# Autodesk Inventor assembly: CockpitLED
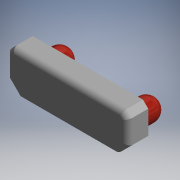
[picture p0: Inventor's stored thumbnail of the model, 180x180]
Saved by Autodesk Inventor 2018.3 (Build 223284000, 284)
## iProperties
Company: A Company
Created: 2018-08-09
Part Number: CockpitLED
Description: KiCad electronic assembly
Document SubType Name: Assembly
Designer: Gregor Gombač
Authority: Unknown
Title: CockpitLED.stp
Author: An Author
Sending System: KiCad to STEP converter
Preprocessor: Open CASCADE STEP processor 6.8
## Documents named in this file (9)
- H:\One Drive Unitn\OneDrive - studenti.unitn.it\FSAE\Schematics\BMS_HV\CockpitLED\CockpitLED.iam
- H:\One Drive Unitn\OneDrive - studenti.unitn.it\FSAE\Schematics\BMS_HV\CockpitLED\C_0805_2012Metric.iam
- H:\One Drive Unitn\OneDrive - studenti.unitn.it\FSAE\Schematics\BMS_HV\CockpitLED\C_1206_3216Metric.iam
- H:\One Drive Unitn\OneDrive - studenti.unitn.it\FSAE\Schematics\BMS_HV\CockpitLED\LED_D10.0mm.iam
- H:\One Drive Unitn\OneDrive - studenti.unitn.it\FSAE\Schematics\BMS_HV\CockpitLED\TSOT-23.iam
- H:\One Drive Unitn\OneDrive - studenti.unitn.it\FSAE\Schematics\BMS_HV\CockpitLED\R_0805_2012Metric.iam
- H:\One Drive Unitn\OneDrive - studenti.unitn.it\FSAE\Schematics\BMS_HV\CockpitLED\R_1206_3216Metric.iam
- H:\One Drive Unitn\OneDrive - studenti.unitn.it\FSAE\Schematics\BMS_HV\CockpitLED\COMPOUND.ipt
- H:\One Drive Unitn\OneDrive - studenti.unitn.it\FSAE\Schematics\BMS_HV\CockpitLED\Box.ipt
## Components (14 placed, 14 different names)
1. 2 [sub-assembly]
2. 4 [sub-assembly]
3. 5 [sub-assembly]
4. 6 [sub-assembly]
5. 8 [sub-assembly]
6. 9 [sub-assembly]
7. 11 [sub-assembly]
8. 12 [sub-assembly]
9. 14 [sub-assembly]
10. 16 [sub-assembly]
11. 17 [sub-assembly]
12. 18 [sub-assembly]
13. 19 — Mate:1, Flush:3, Mate:2
14. Box:1 — Mate:1, Flush:3, Mate:2
## Relationships (3: Mate 2, Flush 1)
- Mate:1: 19 ↔ Box:1
- Flush:3: 19 ↔ Box:1
- Mate:2: 19 ↔ Box:1
